# Autodesk Inventor assembly: rev2 top window wall
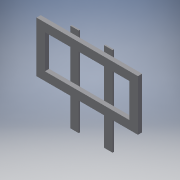
[picture p0: Inventor's stored thumbnail of the model, 180x180]
Saved by Autodesk Inventor 2017 (Build 210142000, 142)
## iProperties
Created: 2019-05-04
Part Number: rev2 top window wall
Document SubType Name: Assembly
Designer: Roman
Author: Roman
## Documents named in this file (4)
- C:\Users\Roman\Documents\CAD\enclosure rev1\rev2 window wall\rev2 top window wall.iam
- C:\Users\Roman\Documents\CAD\enclosure rev1\rev2 window wall\rev2 top window wall h plank.ipt
- C:\Users\Roman\Documents\CAD\enclosure rev1\rev2 window wall\rev2 top window wall v plank.ipt
- C:\Users\Roman\Documents\CAD\enclosure rev1\rev2 base\rev1 beam tube.ipt
## Components (6 placed, 3 different names)
1. rev2 top window wall h plank:1 — Mate:1, Mate:2, Flush:1, Flush:2, Flush:3, Flush:4, Mate:4, Mate:5, Flush:7, Flush:8, Flush:9
2. rev2 top window wall v plank:1 — Mate:1, Flush:2, Flush:3, Mate:3, Flush:5, Flush:6
3. rev2 top window wall v plank:2 — Mate:2, Flush:1, Flush:4, Flush:10
4. rev2 top window wall h plank:2 — Mate:3, Flush:5, Flush:6
5. rev1 beam tube:1 — Mate:4, Flush:8, Flush:9
6. rev1 beam tube:2 — Mate:5, Flush:7, Flush:10
## Relationships (15: Flush 10, Mate 5)
- Mate:1: rev2 top window wall h plank:1 ↔ rev2 top window wall v plank:1
- Mate:2: rev2 top window wall h plank:1 ↔ rev2 top window wall v plank:2
- Flush:1: rev2 top window wall h plank:1 ↔ rev2 top window wall v plank:2
- Flush:2: rev2 top window wall h plank:1 ↔ rev2 top window wall v plank:1
- Flush:3: rev2 top window wall h plank:1 ↔ rev2 top window wall v plank:1
- Flush:4: rev2 top window wall h plank:1 ↔ rev2 top window wall v plank:2
- Mate:3: rev2 top window wall v plank:1 ↔ rev2 top window wall h plank:2
- Flush:5: rev2 top window wall v plank:1 ↔ rev2 top window wall h plank:2
- Flush:6: rev2 top window wall v plank:1 ↔ rev2 top window wall h plank:2
- Mate:4: rev2 top window wall h plank:1 ↔ rev1 beam tube:1
- Mate:5: rev2 top window wall h plank:1 ↔ rev1 beam tube:2
- Flush:7 (-101.6 mm): rev2 top window wall h plank:1 ↔ rev1 beam tube:2
- Flush:8 (-101.6 mm): rev2 top window wall h plank:1 ↔ rev1 beam tube:1
- Flush:9 (533.4 mm): rev2 top window wall h plank:1 ↔ rev1 beam tube:1
- Flush:10 (533.4 mm): rev2 top window wall v plank:2 ↔ rev1 beam tube:2
